# Autodesk Inventor assembly: assemble-s
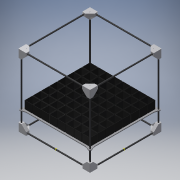
[picture p0: Inventor's stored thumbnail of the model, 180x180]
Saved by Autodesk Inventor 2017 (Build 210142000, 142)
## iProperties
Created: 2019-02-08
Part Number: assemble-s
Document SubType Name: Assembly
Designer: felix
Author: felix
## Documents named in this file (7)
- C:\Users\felix\OneDrive\Documentos\Git\Garatéa E-3\probe-s.iam
- C:\Users\felix\OneDrive\Documentos\Git\Garatéa E-3\probe-s\base.ipt
- C:\Users\felix\OneDrive\Documentos\Git\Garatéa E-3\sats\small_sat.ipt
- C:\Users\felix\OneDrive\Documentos\Git\Garatéa E-3\probe-s\carbon_pipe.ipt
- C:\Users\felix\OneDrive\Documentos\Git\Garatéa E-3\probe-s\connector.ipt
- C:\Users\felix\OneDrive\Documentos\Git\Garatéa E-3\probe-s\connector_MIR.ipt
- C:\Users\felix\OneDrive\Documentos\Git\Garatéa E-3\probe-s\carbon_pipe_MIR.ipt
## Components (85 placed, 6 different names)
1. base:1 — Mate:1, Mate:2, Mate:3, Mate:10
2. small_sat:1 — Mate:1, Mate:2, Mate:3
3. small_sat:2
4. small_sat:3
5. small_sat:4
6. small_sat:5
7. small_sat:6
8. small_sat:7
9. small_sat:8
10. small_sat:9
11. small_sat:10
12. small_sat:11
13. small_sat:12
14. small_sat:13
15. small_sat:14
16. small_sat:15
17. small_sat:16
18. small_sat:17
19. small_sat:18
20. small_sat:19
21. small_sat:20
22. small_sat:21
23. small_sat:22
24. small_sat:23
25. small_sat:24
26. small_sat:25
27. small_sat:26
28. small_sat:27
29. small_sat:28
30. small_sat:29
31. small_sat:30
32. small_sat:31
33. small_sat:32
34. small_sat:33
35. small_sat:34
36. small_sat:35
37. small_sat:36
38. small_sat:37
39. small_sat:38
40. small_sat:39
41. small_sat:40
42. small_sat:41
43. small_sat:42
44. small_sat:43
45. small_sat:44
46. small_sat:45
47. small_sat:46
48. small_sat:47
49. small_sat:48
50. small_sat:49
51. small_sat:50
52. small_sat:51
53. small_sat:52
54. small_sat:53
55. small_sat:54
56. small_sat:55
57. small_sat:56
58. small_sat:57
59. small_sat:58
60. small_sat:59
61. small_sat:60
62. small_sat:61
63. small_sat:62
64. small_sat:63
65. small_sat:64
66. carbon_pipe:2 — Mate:6, Mate:7
67. connector:1 — Mate:4, Mate:5, Mate:6, Mate:7
68. carbon_pipe:1 — Mate:4, Mate:5, Mate:10, Mate:11, Mate:12
69. connector_MIR:1 — Mate:8, Mate:9, Mate:11, Mate:12
70. carbon_pipe_MIR:1 — Mate:8, Mate:9
71. carbon_pipe:3
72. connector:2
73. carbon_pipe:4
74. connector_MIR:2
75. carbon_pipe_MIR:2
76. carbon_pipe:5
77. connector:3
78. carbon_pipe:6
79. connector_MIR:3
80. carbon_pipe_MIR:3
81. carbon_pipe:7
82. connector:4
83. carbon_pipe:8
84. connector_MIR:4
85. carbon_pipe_MIR:4
## Component patterns: (64 elements, first: small_sat:1), (4 elements, first: carbon_pipe:2 + connector:1 + carbon_pipe:1 + connector_MIR:1 + carbon_pipe_MIR:1)
## Relationships (12: Mate 12)
- Mate:1: base:1 ↔ small_sat:1
- Mate:2: base:1 ↔ small_sat:1
- Mate:3: base:1 ↔ small_sat:1
- Mate:4: connector:1 ↔ carbon_pipe:1
- Mate:5: connector:1 ↔ carbon_pipe:1
- Mate:6: carbon_pipe:2 ↔ connector:1
- Mate:7: carbon_pipe:2 ↔ connector:1
- Mate:8: connector_MIR:1 ↔ carbon_pipe_MIR:1
- Mate:9: connector_MIR:1 ↔ carbon_pipe_MIR:1
- Mate:10: base:1 ↔ carbon_pipe:1
- Mate:11: carbon_pipe:1 ↔ connector_MIR:1
- Mate:12: carbon_pipe:1 ↔ connector_MIR:1
